# Autodesk Inventor assembly: 10mm_cnc_v1
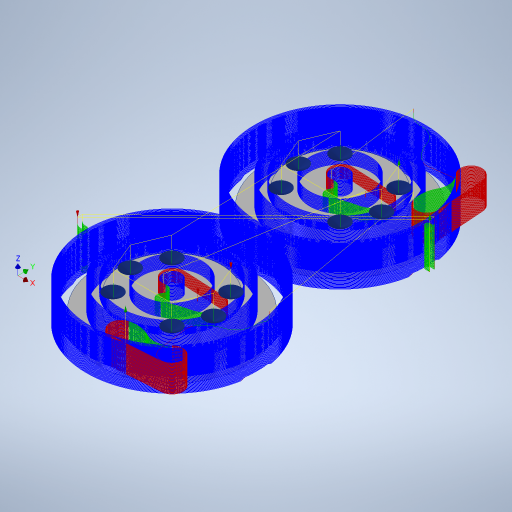
[picture p0: Inventor's stored thumbnail of the model, 512x512]
Saved by Autodesk Inventor 2024 (Build 280153000, 153)
## iProperties
Created: 2025-07-12
Part Number: 10mm_cnc_v1
Document SubType Name: Assembly
Designer: tanoue_kota
Author: tanoue_kota
## Documents named in this file (2)
- C:\Users\田之上巧太\Documents\Create_ViperX_ALOHA\FlatPattern\10mm_cnc_v1.iam
- C:\Users\田之上巧太\Documents\Create_ViperX_ALOHA\ForeArm_Component\connectpart2.ipt
## Components (2 placed, 1 different names)
1. connectpart2:1 — フラッシュ:1
2. connectpart2:2 — フラッシュ:1
## Relationships (1: Flush 1)
- フラッシュ:1 [Flush]: connectpart2:1 ↔ connectpart2:2
